# Autodesk Inventor assembly: 000 Ensamblaje 3d_LM - BASIC
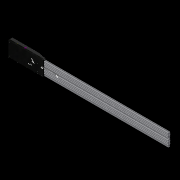
[picture p0: Inventor's stored thumbnail of the model, 180x180]
Saved by Autodesk Inventor 2018.3 (Build 223284000, 284)
## iProperties
Category: 0
Created: 2025-11-12
Part Number: 000 Ensamblaje 3d_LM - BASIC
Document SubType Name: Assembly
Designer: mbs18
Mass: 1075.01 g
Surface Area: 1597.09 cm^2
Volume: 206.309 cm^3
Density: 5.21067 g/cm^3
Manufacturer-1: {"Link": "", "Name": "\nEmbention Sistemas Inteligentes S.A.", "PartNumber": "3d_LM - BASIC", "partner_id": false}
Manufacturer-2: {"Link": "", "Name": "", "PartNumber": "", "partner_id": false}
Manufacturer-3: {"Link": "", "Name": "", "PartNumber": "", "partner_id": false}
Manufacturer-4: {"Link": "", "Name": "", "PartNumber": "", "partner_id": false}
Manufacturer-5: {"Link": "", "Name": "", "PartNumber": "", "partner_id": false}
Provider-1: {"Link": "", "Name": "", "PartNumber": "", "partner_id": false}
Provider-2: {"Link": "", "Name": "", "PartNumber": "", "partner_id": false}
Provider-3: {"Link": "", "Name": "", "PartNumber": "", "partner_id": false}
Provider-4: {"Link": "", "Name": "", "PartNumber": "", "partner_id": false}
Provider-5: {"Link": "", "Name": "", "PartNumber": "", "partner_id": false}
odoo_id: 19225
odoo_item_code: 3d_LM
odoo_internal_code: P015262
odoo_pt_internal_code: PT12060
odoo_part_number_code: 3d_LM/BASIC-101010
odoo_model: product.template
odoo_x2o_application_version: 12.0.4.20
odoo_d2o_version: 12.0.1.6.0
Author: mbs18
## Documents named in this file (13)
- C:\Users\mbs18.Embention\Git\LM\items\3d_LM\variants\BASIC\000 Ensamblaje 3d_LM - BASIC.iam
- C:\Users\mbs18.Embention\Git\LM\items\3d_LM\hw_LM\3d\000 Ensamblaje hw_LM - BASIC.iam
- C:\Users\mbs18.Embention\Git\LM\items\3d_LM\3d\3d_LM - Tubo 1x1.ipt
- C:\Users\mbs18.Embention\Git\LM\items\3d_LM\variants\BASIC\000 Ensamblaje 3d_LM - BASIC\AIP\Cable and Harness\000 Ensamblaje 3d_LM - BASIC.Harness1.iam
- C:\Users\mbs18.Embention\Git\LM\items\_accesories\Cables y conectores\3d_Hirose Electric Co Ltd\3d\UFL\U_FL-LP-066HF.ipt
- C:\Users\mbs18.Embention\Git\LM\items\_accesories\Tornilleria\Tornillos\3d_ISO 7380\3d\A2 Inox\SSB-M2.5-5-A2.ipt
- C:\Users\mbs18.Embention\Git\LM\items\3d_LM\3d\3d_LM - Pinza 3.ipt
- C:\Users\mbs18.Embention\Git\LM\items\3d_LM\3d\3d_LM - Pinza 2.ipt
- C:\Users\mbs18.Embention\Git\LM\items\3d_LM\3d\3d_LM - Pinza 1.ipt
- C:\Users\mbs18.Embention\Git\LM\items\3d_LM\3d\3d_LM - Pinza 4.ipt
- C:\Users\mbs18.Embention\Git\LM\items\3d_LM\3d\3d_LM - Bottom Wire.ipt
- C:\Users\mbs18.Embention\Git\LM\items\3d_LM\3d\3d_LM - Top Wire.ipt
- C:\Users\mbs18.Embention\Git\LM\items\3d_LM\3d\3d_LM - Cover.ipt
## Components (15 placed, 12 different names)
1. 3d_LM - Cover:1 — Mate:3, Mate:4, Flush:36, Flush:37
2. 3d_LM - Pinza 3:1 — Mate:108, Mate:109, Mate:110, Mate:111, Mate:112, Flush:35, Mate:114
3. 3d_LM - Pinza 2:1 — Flush:31, Mate:97, Mate:98, Angle:2, Mate:104, Mate:106, Mate:109, Mate:113, Flush:36, Flush:37, Flush:38
4. 3d_LM - Pinza 1:1 — Flush:31, Mate:97, Mate:98
5. 3d_LM - Pinza 4:1 — Mate:102, Mate:103, Mate:108
6. 3d_LM - Tubo 1x1:1 — Flush:34, Mate:113
7. 3d_LM - Tubo 1x1:2 — Mate:106, Flush:34, Mate:115
8. U_FL-LP-066HF:2 — Mate:56, Flush:29
9. U_FL-LP-066HF:1 — Mate:58, Flush:28
10. 3d_LM - Bottom Wire:1 — Mate:102, Mate:103, Flush:33, Mate:111
11. 3d_LM - Top Wire:1 — Mate:104, Flush:33, Mate:110, Mate:114, Flush:38
12. Harness1 [sub-assembly]
13. SSB-M2.5-5-A2:1 — Mate:60, Mate:61
14. SSB-M2.5-5-A2:2 — Mate:63, Mate:69
15. 000 Ensamblaje hw_LM - BASIC:1 [sub-assembly] — Mate:1, Flush:1, Mate:2, Mate:4, Mate:56, Mate:58, Mate:60, Mate:61, Mate:63, Mate:69, Flush:28, Flush:29, Angle:2, Mate:112, Flush:35, Mate:115
## Relationships (35: Mate 24, Flush 10, Angle 1)
- Mate:1: 000 Ensamblaje hw_LM - BASIC:1
- Flush:1: 000 Ensamblaje hw_LM - BASIC:1
- Mate:2: 000 Ensamblaje hw_LM - BASIC:1
- Mate:3: 3d_LM - Cover:1
- Mate:4 (4.7 mm): 3d_LM - Cover:1 ↔ 000 Ensamblaje hw_LM - BASIC:1
- Mate:56: U_FL-LP-066HF:2 ↔ 000 Ensamblaje hw_LM - BASIC:1
- Mate:58: U_FL-LP-066HF:1 ↔ 000 Ensamblaje hw_LM - BASIC:1
- Mate:60: SSB-M2.5-5-A2:1 ↔ 000 Ensamblaje hw_LM - BASIC:1
- Mate:61: SSB-M2.5-5-A2:1 ↔ 000 Ensamblaje hw_LM - BASIC:1
- Mate:63: SSB-M2.5-5-A2:2 ↔ 000 Ensamblaje hw_LM - BASIC:1
- Mate:69: SSB-M2.5-5-A2:2 ↔ 000 Ensamblaje hw_LM - BASIC:1
- Flush:28 (-2.5 mm): U_FL-LP-066HF:1 ↔ 000 Ensamblaje hw_LM - BASIC:1
- Flush:29 (-3.2 mm): U_FL-LP-066HF:2 ↔ 000 Ensamblaje hw_LM - BASIC:1
- Flush:31: 3d_LM - Pinza 2:1 ↔ 3d_LM - Pinza 1:1
- Mate:97: 3d_LM - Pinza 2:1 ↔ 3d_LM - Pinza 1:1
- Mate:98: 3d_LM - Pinza 2:1 ↔ 3d_LM - Pinza 1:1
- Angle:2 (0 deg): 3d_LM - Pinza 2:1 ↔ 000 Ensamblaje hw_LM - BASIC:1
- Mate:102: 3d_LM - Pinza 4:1 ↔ 3d_LM - Bottom Wire:1
- Mate:103: 3d_LM - Pinza 4:1 ↔ 3d_LM - Bottom Wire:1
- Mate:104: 3d_LM - Pinza 2:1 ↔ 3d_LM - Top Wire:1
- Flush:33: 3d_LM - Bottom Wire:1 ↔ 3d_LM - Top Wire:1
- Mate:106: 3d_LM - Pinza 2:1 ↔ 3d_LM - Tubo 1x1:2
- Flush:34: 3d_LM - Tubo 1x1:1 ↔ 3d_LM - Tubo 1x1:2
- Mate:108: 3d_LM - Pinza 3:1 ↔ 3d_LM - Pinza 4:1
- Mate:109: 3d_LM - Pinza 3:1 ↔ 3d_LM - Pinza 2:1
- Mate:110: 3d_LM - Pinza 3:1 ↔ 3d_LM - Top Wire:1
- Mate:111: 3d_LM - Pinza 3:1 ↔ 3d_LM - Bottom Wire:1
- Mate:112: 3d_LM - Pinza 3:1 ↔ 000 Ensamblaje hw_LM - BASIC:1
- Flush:35 (-0.25 mm): 3d_LM - Pinza 3:1 ↔ 000 Ensamblaje hw_LM - BASIC:1
- Mate:113: 3d_LM - Pinza 2:1 ↔ 3d_LM - Tubo 1x1:1
- Flush:36 (1 mm): 3d_LM - Cover:1 ↔ 3d_LM - Pinza 2:1
- Flush:37 (-5 mm): 3d_LM - Cover:1 ↔ 3d_LM - Pinza 2:1
- Mate:114: 3d_LM - Pinza 3:1 ↔ 3d_LM - Top Wire:1
- Flush:38 (-1 mm): 3d_LM - Pinza 2:1 ↔ 3d_LM - Top Wire:1
- Mate:115: 3d_LM - Tubo 1x1:2 ↔ 000 Ensamblaje hw_LM - BASIC:1
